# Autodesk Inventor assembly: recuperation
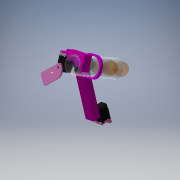
[picture p0: Inventor's stored thumbnail of the model, 180x180]
Saved by Autodesk Inventor 2017 (Build 210142000, 142)
## iProperties
Created: 2018-03-31
Part Number: recuperation
Document SubType Name: Assembly
Designer: franc
Mass: 446.753 g
Surface Area: 1710.63 cm^2
Volume: 446.753 cm^3
Density: 1 g/cm^3
Author: franc
## Documents named in this file (13)
- C:\Users\franc\Desktop\EsialRobotik\Mecanique\2018\robot\traitement-eau\recuperation.iam
- C:\Users\franc\Desktop\EsialRobotik\Mecanique\2018\robot\traitement-eau\cylindre-stockage.ipt
- C:\Users\franc\Desktop\EsialRobotik\Mecanique\2018\robot\traitement-eau\eau.ipt
- C:\Users\franc\Desktop\EsialRobotik\Mecanique\composants\AX12\AX12.iam
- C:\Users\franc\Desktop\EsialRobotik\Mecanique\2018\robot\traitement-eau\trappe.ipt
- C:\Users\franc\Desktop\EsialRobotik\Mecanique\composants\AX12\F3.ipt
- C:\Users\franc\Desktop\EsialRobotik\Mecanique\2018\robot\traitement-eau\support-trappe.ipt
- C:\Users\franc\Desktop\EsialRobotik\Mecanique\composants\AX12\F2.ipt
- C:\Users\franc\Desktop\EsialRobotik\Mecanique\composants\AX12\ax12_wheel.ipt
- C:\Users\franc\Desktop\EsialRobotik\Mecanique\composants\AX12\ax12_box.ipt
- C:\Users\franc\Desktop\EsialRobotik\Mecanique\2018\robot\traitement-eau\rotation-recuperation.ipt
- C:\Users\franc\Desktop\EsialRobotik\Mecanique\2018\robot\traitement-eau\bras.ipt
- C:\Users\franc\Desktop\EsialRobotik\Mecanique\2018\robot\traitement-eau\fixation-bras.ipt
## Components (16 placed, 12 different names)
1. cylindre-stockage:1 — Placage:1, Placage:2, Placage:3, Placage:4, Affleurement:1, Tangente:7, Tangente:8, Tangente:9, Affleurement:3, Placage:22, Tangente:11
2. eau:1 — Placage:1, Tangente:11, Tangente:12
3. eau:2 — Placage:2, Tangente:12, Tangente:13
4. eau:3 — Placage:3, Tangente:13, Tangente:14
5. eau:4 — Placage:4, Tangente:14
6. AX12:1 [sub-assembly] — Affleurement:1, Tangente:5, Tangente:6, Placage:5, Placage:6, Placage:7, Placage:8, Tangente:7, Tangente:8
7. trappe:1 — Tangente:5, Tangente:6, Placage:5
8. F3:1 — Placage:6, Placage:7, Placage:8, Placage:9, Affleurement:2, Placage:10
9. support-trappe:1 — Placage:9, Affleurement:2, Placage:10, Affleurement:4
10. F2:1 — Placage:11, Placage:12, Placage:13, Tangente:9, Affleurement:3, Affleurement:4, Placage:14, Affleurement:5
11. ax12_wheel:1 — Placage:11, Placage:12, Placage:13
12. ax12_box:1 — Placage:15, Placage:16, Placage:17
13. rotation-recuperation:1 — Placage:14, Affleurement:5, Placage:22
14. bras:1 — Placage:15, Placage:16, Placage:17, Placage:18, Affleurement:6, Tangente:10
15. AX12:2 [sub-assembly] — Placage:18, Affleurement:6, Tangente:10, Placage:19, Placage:20, Placage:21
16. fixation-bras:1 — Placage:19, Placage:20, Placage:21
## Relationships (39: Mate 22, Tangent 10, Flush 6, Insert 1)
- Placage:1 [Mate]: cylindre-stockage:1 ↔ eau:1
- Placage:2 [Mate]: cylindre-stockage:1 ↔ eau:2
- Placage:3 [Mate]: cylindre-stockage:1 ↔ eau:3
- Placage:4 [Mate]: cylindre-stockage:1 ↔ eau:4
- Affleurement:1 [Flush]: cylindre-stockage:1 ↔ AX12:1
- Tangente:5: AX12:1 ↔ trappe:1
- Tangente:6: AX12:1 ↔ trappe:1
- Placage:5 [Mate]: AX12:1 ↔ trappe:1
- Placage:6 [Mate]: AX12:1 ↔ F3:1
- Placage:7 [Mate]: AX12:1 ↔ F3:1
- Placage:8 [Mate]: AX12:1 ↔ F3:1
- Tangente:7 (1 mm): cylindre-stockage:1 ↔ AX12:1
- Tangente:8: cylindre-stockage:1 ↔ AX12:1
- Placage:9 [Mate]: F3:1 ↔ support-trappe:1
- Affleurement:2 [Flush]: F3:1 ↔ support-trappe:1
- Placage:10 [Mate]: F3:1 ↔ support-trappe:1
- [Insert]: ax12_wheel:1 ↔ ax12_box:1
- Placage:11 [Mate]: F2:1 ↔ ax12_wheel:1
- Placage:12 [Mate]: F2:1 ↔ ax12_wheel:1
- Placage:13 [Mate]: F2:1 ↔ ax12_wheel:1
- Tangente:9 (1 mm): cylindre-stockage:1 ↔ F2:1
- Affleurement:3 [Flush] (87.5 mm): cylindre-stockage:1 ↔ F2:1
- Affleurement:4 [Flush] (25.5 mm): support-trappe:1 ↔ F2:1
- Placage:14 [Mate]: F2:1 ↔ rotation-recuperation:1
- Affleurement:5 [Flush]: F2:1 ↔ rotation-recuperation:1
- Placage:15 [Mate]: ax12_box:1 ↔ bras:1
- Placage:16 [Mate]: ax12_box:1 ↔ bras:1
- Placage:17 [Mate]: ax12_box:1 ↔ bras:1
- Placage:18 [Mate]: bras:1 ↔ AX12:2
- Affleurement:6 [Flush] (-23.5 mm): bras:1 ↔ AX12:2
- Tangente:10 (6 mm): bras:1 ↔ AX12:2
- Placage:19 [Mate]: AX12:2 ↔ fixation-bras:1
- Placage:20 [Mate]: AX12:2 ↔ fixation-bras:1
- Placage:21 [Mate]: AX12:2 ↔ fixation-bras:1
- Placage:22 [Mate]: cylindre-stockage:1 ↔ rotation-recuperation:1
- Tangente:11: cylindre-stockage:1 ↔ eau:1
- Tangente:12: eau:1 ↔ eau:2
- Tangente:13: eau:2 ↔ eau:3
- Tangente:14: eau:3 ↔ eau:4
## Named parameters: d28_d1 = 0 mm
